# Autodesk Inventor assembly: small-model-rocket-launch-pad
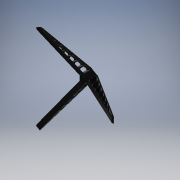
[picture p0: Inventor's stored thumbnail of the model, 180x180]
Saved by Autodesk Inventor 2017 (Build 210142000, 142)
## iProperties
Created: 2020-06-17
Part Number: small-model-rocket-launch-pad
Document SubType Name: Assembly
Designer: HAYNIE R&D
Author: HAYNIE R&D
## Documents named in this file (3)
- C:\Users\HAYNIE\source\repos\small-model-rocket-launch-pad\small-model-rocket-launch-pad.iam
- C:\Users\HAYNIE\source\repos\small-model-rocket-launch-pad\center.ipt
- C:\Users\HAYNIE\source\repos\small-model-rocket-launch-pad\leg.ipt
## Components (4 placed, 2 different names)
1. center:1 — Slider:2, Slider:4, Slider:5
2. leg:1 — Slider:2
3. leg:2 — Slider:5
4. leg:3 — Slider:4
## Relationships (3: TranslationJoint 3)
- Slider:2 [TranslationJoint]: center:1 ↔ leg:1
- Slider:4 [TranslationJoint]: center:1 ↔ leg:3
- Slider:5 [TranslationJoint]: center:1 ↔ leg:2
